# Autodesk Inventor assembly: ASY Disk Micro filter v2.0
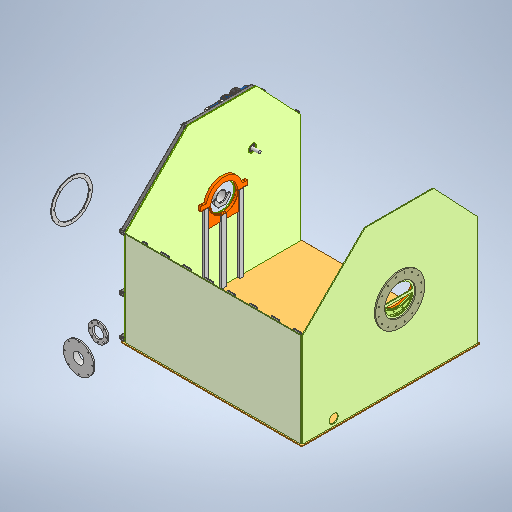
[picture p0: Inventor's stored thumbnail of the model, 512x512]
Saved by Autodesk Inventor 2025 (Build 290162010, 162A)
## iProperties
Created: 2023-08-31
Part Number: ASY Disk Micro filter v2.0
Document SubType Name: Assembly
Designer: admin
Stock Number: Дисковый_Фильтр
Author: admin
## Documents named in this file (36)
- C:\Users\pokla\Documents\Inventor\ДФО\ДМФ\DMF-Disk-Micro-Filter\ASY 000 ДМФ Disk Micro filter v2.0.iam
- C:\Users\pokla\Documents\Inventor\ДФО\ДМФ\DMF-Disk-Micro-Filter\Left wall v2.0.ipt
- C:\Users\pokla\Documents\Inventor\ДФО\ДМФ\DMF-Disk-Micro-Filter\Wall right v2.0.ipt
- C:\Users\pokla\Documents\Inventor\ДФО\ДМФ\DMF-Disk-Micro-Filter\DF1.03 Wall bottom v2.0.ipt
- C:\Users\pokla\Documents\Inventor\ДФО\ДМФ\DMF-Disk-Micro-Filter\DF1.04 Wall face v2.0.ipt
- C:\Users\pokla\Documents\Inventor\ДФО\ДМФ\DMF-Disk-Micro-Filter\ДМФ 021 кольцо прижимное нос v2.0.ipt
- C:\Users\pokla\Documents\Inventor\ДФО\ДМФ\DMF-Disk-Micro-Filter\ДМФ 000 размеры v2.0.ipt
- C:\Users\pokla\Documents\Inventor\ДФО\ДМФ\DMF-Disk-Micro-Filter\ДМФ 032 крышка Нос v2.0.ipt
- C:\Users\pokla\Documents\Inventor\ДФО\ДМФ\DMF-Disk-Micro-Filter\ДМФ 091 Постель НОС v2.0.ipt
- C:\Users\pokla\Documents\Inventor\ДФО\ДМФ\DMF-Disk-Micro-Filter\ДМФ 022 кольцо прижимное корма v2.0.ipt
- C:\Users\pokla\Documents\Inventor\ДФО\ДМФ\DMF-Disk-Micro-Filter\ДМФ 093 Постель КОРМА v2.0.ipt
- C:\Users\pokla\Documents\Inventor\ДФО\ДМФ\DMF-Disk-Micro-Filter\ДМФ 092 Коромысло КОРМА v2.0.ipt
- C:\Users\pokla\Documents\Inventor\ДФО\ДМФ\DMF-Disk-Micro-Filter\ДМФ 055 труба илоотвода v2.0.ipt
- C:\Users\pokla\Documents\Inventor\ДФО\ДМФ\DMF-Disk-Micro-Filter\ДМФ 033 держатель лотка v2.0.ipt
- C:\Users\pokla\Documents\Inventor\ДФО\ДМФ\DMF-Disk-Micro-Filter\ASY ДМФ лоток 050 илоотвод v2.0.iam
- C:\Users\pokla\Documents\Inventor\ДФО\ДМФ\DMF-Disk-Micro-Filter\ДМФ 092 Коромысло НОС v2.0.ipt
- C:\Users\pokla\Documents\Inventor\ДФО\ДМФ\DMF-Disk-Micro-Filter\ДМФ 011 Стенка Корма ЛЕВ v2.0.ipt
- C:\Users\pokla\Documents\Inventor\ДФО\ДМФ\DMF-Disk-Micro-Filter\ДМФ 012 Стенка Корма ПРАВ v2.0.ipt
- C:\Users\pokla\Documents\Inventor\ДФО\ДМФ\DMF-Disk-Micro-Filter\ДМФ 014 Стенка Нос ЛЕВ v2.0.ipt
- C:\Users\pokla\Documents\Inventor\ДФО\ДМФ\DMF-Disk-Micro-Filter\ДМФ 015 Стенка Нос ПРАВ v2.0.ipt
- C:\Users\pokla\Documents\Inventor\ДФО\ДМФ\DMF-Disk-Micro-Filter\ДМФ 066 Гребенка v2.0.ipt
- C:\Users\pokla\Documents\Inventor\ДФО\ДМФ\DMF-Disk-Micro-Filter\ДМФ 025 кольцо прижимное корма наружное v2.0.ipt
- C:\Users\pokla\Documents\Inventor\ДФО\ДМФ\DMF-Disk-Micro-Filter\ДМФ 067 крышка v2.0.ipt
- C:\Users\pokla\Documents\Inventor\ДФО\ДМФ\DMF-Disk-Micro-Filter\ДМФ 081 труба форсунки v2.0.ipt
- C:\Users\pokla\Documents\Inventor\ДФО\ДМФ\DMF-Disk-Micro-Filter\ASY Обрешетка лицевая стенка.iam
- C:\Users\pokla\Documents\Inventor\ДФО\ДМФ\DMF-Disk-Micro-Filter\ASY Консоль под двигатель вед. шестерни.iam
- C:\Users\pokla\Documents\Inventor\ДФО\ДМФ\DMF-Disk-Micro-Filter\Вал ведущей шестерни.ipt
- C:\Users\pokla\Documents\Inventor\ДФО\ДМФ\DMF-Disk-Micro-Filter\Корпусный подшипник D35.ipt
- C:\Users\pokla\Documents\Inventor\ДФО\ДМФ\DMF-Disk-Micro-Filter\Мотор-редуктор NMRV 090(80B5).ipt
- C:\Users\pokla\Documents\Inventor\ДФО\ДМФ\DMF-Disk-Micro-Filter\Кольцо проект Алексенко.ipt
- C:\Users\pokla\Documents\Inventor\ДФО\ДМФ\DMF-Disk-Micro-Filter\Нога для постели.ipt
- C:\Users\pokla\Documents\Inventor\ДФО\ДМФ\DMF-Disk-Micro-Filter\Нога для постели №2.ipt
- C:\Users\pokla\Documents\Inventor\ДФО\ДМФ\DMF-Disk-Micro-Filter\ДМФ 092 Постель НОС v2.0.ipt
- C:\Users\pokla\Documents\Inventor\ДФО\ДМФ\DMF-Disk-Micro-Filter\ДМФ 094 Постель НОС крепление v2.0.ipt
- C:\Users\pokla\Documents\Inventor\ДФО\ДМФ\DMF-Disk-Micro-Filter\DMF Hat 2.0.ipt
- C:\Users\pokla\Documents\Inventor\ДФО\ДМФ\DMF-Disk-Micro-Filter\DMF Flange exit 2.0.ipt
## Components (37 placed, 35 different names)
1. ДМФ 000 размеры v2.0.ipt:1
2. Left wall v2.0.ipt:1 — Flush:4, Mate:1, Flush:6, Flush:7, Flush:9, Mate:4, Rotational:12, Rigid:12, Flush:26, Flush:27, Mate:25, Rigid:16, Mate:29, Rigid:22
3. Wall right v2.0.ipt:1 — Mate:22, Rigid:14, Flush:23, Flush:24, Rigid:16
4. DF1.03 Wall bottom v2.0.ipt:1 — Mate:1, Flush:6, Flush:7, Mate:3, Flush:11, Mate:24, Mate:30
5. DF1.04 Wall face v2.0.ipt:1 — Flush:9, Mate:3, Mate:4, Flush:10, Angle:1
6. ДМФ 021 кольцо прижимное нос v2.0.ipt:1 — Rotational:12, Mate:13
7. ДМФ 032 крышка Нос v2.0.ipt:1 — Mate:16, Rigid:8, Rigid:12
8. ДМФ 091 Постель НОС v2.0.ipt:1 — Rigid:18, Rigid:19, Rigid:20, Rigid:25
9. ДМФ 022 кольцо прижимное корма v2.0.ipt:1 — Flush:18, Rigid:11
10. ДМФ 093 Постель КОРМА v2.0.ipt:1 — Mate:15, Rigid:3, Rigid:11
11. ДМФ 092 Коромысло КОРМА v2.0.ipt:1 — Rigid:3
12. ДМФ 055 труба илоотвода v2.0.ipt:1 — Rigid:8, Tangent:1
13. ДМФ 033 держатель лотка v2.0.ipt:1 — Mate:16, Mate:17, Tangent:1, Mate:23
14. ASY ДМФ лоток 050 илоотвод v2.0.iam:1 [sub-assembly] — Mate:22, Mate:23
15. ДМФ 092 Коромысло НОС v2.0.ipt:1 — Rigid:21, Rigid:22
16. ДМФ 011 Стенка Корма ЛЕВ v2.0.ipt:1
17. ДМФ 012 Стенка Корма ПРАВ v2.0.ipt:1
18. ДМФ 014 Стенка Нос ЛЕВ v2.0.ipt:1
19. ДМФ 015 Стенка Нос ПРАВ v2.0.ipt:1
20. ДМФ 066 Гребенка v2.0.ipt:1 — Flush:22, Angle:1, Mate:24
21. ДМФ 025 кольцо прижимное корма наружное v2.0.ipt:1 — Rigid:14
22. ДМФ 067 крышка v2.0.ipt:1 — Flush:23, Flush:24, Flush:25, Rotational:16
23. ДМФ 081 труба форсунки v2.0.ipt:1 — Flush:25, Rotational:16
24. ASY Обрешетка лицевая стенка.iam:1 [sub-assembly] — Flush:26, Flush:27, Mate:25, Mate:26, Flush:28, Mate:27, Flush:29, Flush:30
25. ASY Консоль под двигатель вед. шестерни.iam:1 [sub-assembly] — Mate:26, Flush:28, Flush:30, Mate:28, Flush:31
26. Вал ведущей шестерни:1 — Rotational:18
27. Корпусный подшипник D35:1 — Mate:27, Flush:29, Rotational:18
28. Мотор-редуктор NMRV 090(80B5):1 — Mate:28, Flush:31
29. Кольцо проект Алексенко:1
30. Нога для постели:1 — Rigid:23
31. Нога для постели:2 — Rigid:24
32. Нога для постели №2:1 — Mate:29, Rigid:25
33. ДМФ 092 Постель НОС v2.0:1 — Rigid:18
34. ДМФ 094 Постель НОС крепление v2.0:1 — Rigid:19, Rigid:21, Rigid:24
35. ДМФ 094 Постель НОС крепление v2.0:2 — Rigid:20, Rigid:23
36. DMF Hat 2.0:1
37. DMF Flange exit 2.0:1
## Relationships (53: Flush 17, Mate 17, WeldJoint 14, RevoluteJoint 3, Tangent 1, Angle 1)
- Flush:4: Left wall v2.0.ipt:1
- Mate:1: Left wall v2.0.ipt:1 ↔ DF1.03 Wall bottom v2.0.ipt:1
- Flush:6 (15 mm): Left wall v2.0.ipt:1 ↔ DF1.03 Wall bottom v2.0.ipt:1
- Flush:7 (25 mm): Left wall v2.0.ipt:1 ↔ DF1.03 Wall bottom v2.0.ipt:1
- Flush:9: Left wall v2.0.ipt:1 ↔ DF1.04 Wall face v2.0.ipt:1
- Mate:3: DF1.03 Wall bottom v2.0.ipt:1 ↔ DF1.04 Wall face v2.0.ipt:1
- Mate:4: Left wall v2.0.ipt:1 ↔ DF1.04 Wall face v2.0.ipt:1
- Flush:10: DF1.04 Wall face v2.0.ipt:1
- Flush:11: DF1.03 Wall bottom v2.0.ipt:1
- Rotational:12 [RevoluteJoint]: Left wall v2.0.ipt:1 ↔ ДМФ 021 кольцо прижимное нос v2.0.ipt:1
- Mate:13: ДМФ 021 кольцо прижимное нос v2.0.ipt:1
- Flush:18: ДМФ 022 кольцо прижимное корма v2.0.ipt:1
- Mate:15: ДМФ 093 Постель КОРМА v2.0.ipt:1
- Rigid:3 [WeldJoint]: ДМФ 093 Постель КОРМА v2.0.ipt:1 ↔ ДМФ 092 Коромысло КОРМА v2.0.ipt:1
- [Mate]: ASY ДМФ лоток 050 илоотвод v2.0.iam:1
- Mate:16: ДМФ 032 крышка Нос v2.0.ipt:1 ↔ ДМФ 033 держатель лотка v2.0.ipt:1
- Mate:17: ДМФ 033 держатель лотка v2.0.ipt:1
- Rigid:8 [WeldJoint]: ДМФ 032 крышка Нос v2.0.ipt:1 ↔ ДМФ 055 труба илоотвода v2.0.ipt:1
- Tangent:1: ДМФ 055 труба илоотвода v2.0.ipt:1 ↔ ДМФ 033 держатель лотка v2.0.ipt:1
- Mate:22: Wall right v2.0.ipt:1 ↔ ASY ДМФ лоток 050 илоотвод v2.0.iam:1
- Mate:23: ДМФ 033 держатель лотка v2.0.ipt:1 ↔ ASY ДМФ лоток 050 илоотвод v2.0.iam:1
- Rigid:11 [WeldJoint]: ДМФ 022 кольцо прижимное корма v2.0.ipt:1 ↔ ДМФ 093 Постель КОРМА v2.0.ipt:1
- Rigid:12 [WeldJoint]: Left wall v2.0.ipt:1 ↔ ДМФ 032 крышка Нос v2.0.ipt:1
- Flush:22: ДМФ 066 Гребенка v2.0.ipt:1
- Angle:1 (180 deg): DF1.04 Wall face v2.0.ipt:1 ↔ ДМФ 066 Гребенка v2.0.ipt:1
- Mate:24: DF1.03 Wall bottom v2.0.ipt:1 ↔ ДМФ 066 Гребенка v2.0.ipt:1
- Rigid:14 [WeldJoint]: Wall right v2.0.ipt:1 ↔ ДМФ 025 кольцо прижимное корма наружное v2.0.ipt:1
- Flush:23: Wall right v2.0.ipt:1 ↔ ДМФ 067 крышка v2.0.ipt:1
- Flush:24 (-50 mm): Wall right v2.0.ipt:1 ↔ ДМФ 067 крышка v2.0.ipt:1
- Flush:25: ДМФ 067 крышка v2.0.ipt:1 ↔ ДМФ 081 труба форсунки v2.0.ipt:1
- Rotational:16 [RevoluteJoint]: ДМФ 067 крышка v2.0.ipt:1 ↔ ДМФ 081 труба форсунки v2.0.ipt:1
- Flush:26: Left wall v2.0.ipt:1 ↔ ASY Обрешетка лицевая стенка.iam:1
- Flush:27: Left wall v2.0.ipt:1 ↔ ASY Обрешетка лицевая стенка.iam:1
- Mate:25: Left wall v2.0.ipt:1 ↔ ASY Обрешетка лицевая стенка.iam:1
- Mate:26: ASY Обрешетка лицевая стенка.iam:1 ↔ ASY Консоль под двигатель вед. шестерни.iam:1
- Flush:28: ASY Обрешетка лицевая стенка.iam:1 ↔ ASY Консоль под двигатель вед. шестерни.iam:1
- Rigid:16 [WeldJoint] (2160 mm): Left wall v2.0.ipt:1 ↔ Wall right v2.0.ipt:1
- Mate:27: ASY Обрешетка лицевая стенка.iam:1 ↔ Корпусный подшипник D35:1
- Flush:29 (1 mm): ASY Обрешетка лицевая стенка.iam:1 ↔ Корпусный подшипник D35:1
- Rotational:18 [RevoluteJoint] (-359.5 mm): Вал ведущей шестерни:1 ↔ Корпусный подшипник D35:1
- Flush:30: ASY Обрешетка лицевая стенка.iam:1 ↔ ASY Консоль под двигатель вед. шестерни.iam:1
- Mate:28: ASY Консоль под двигатель вед. шестерни.iam:1 ↔ Мотор-редуктор NMRV 090(80B5):1
- Flush:31: ASY Консоль под двигатель вед. шестерни.iam:1 ↔ Мотор-редуктор NMRV 090(80B5):1
- Mate:29: Left wall v2.0.ipt:1 ↔ Нога для постели №2:1
- Mate:30: DF1.03 Wall bottom v2.0.ipt:1
- Rigid:18 [WeldJoint]: ДМФ 091 Постель НОС v2.0.ipt:1 ↔ ДМФ 092 Постель НОС v2.0:1
- Rigid:19 [WeldJoint]: ДМФ 091 Постель НОС v2.0.ipt:1 ↔ ДМФ 094 Постель НОС крепление v2.0:1
- Rigid:20 [WeldJoint]: ДМФ 091 Постель НОС v2.0.ipt:1 ↔ ДМФ 094 Постель НОС крепление v2.0:2
- Rigid:21 [WeldJoint]: ДМФ 092 Коромысло НОС v2.0.ipt:1 ↔ ДМФ 094 Постель НОС крепление v2.0:1
- Rigid:22 [WeldJoint]: Left wall v2.0.ipt:1 ↔ ДМФ 092 Коромысло НОС v2.0.ipt:1
- Rigid:23 [WeldJoint]: Нога для постели:1 ↔ ДМФ 094 Постель НОС крепление v2.0:2
- Rigid:24 [WeldJoint]: Нога для постели:2 ↔ ДМФ 094 Постель НОС крепление v2.0:1
- Rigid:25 [WeldJoint]: ДМФ 091 Постель НОС v2.0.ipt:1 ↔ Нога для постели №2:1
